# Autodesk Inventor assembly: magplate_blank
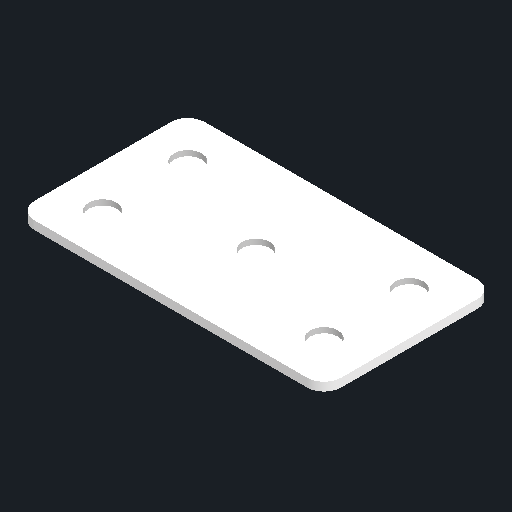
[picture p0: Inventor's stored thumbnail of the model, 512x512]
Saved by Autodesk Inventor 2025 (Build 290162000, 162)
## iProperties
Created: 2024-06-22
Part Number: magplate_blank
Document SubType Name: Assembly
Designer: AdminForWorker
Title: magplate_blank v6
Author: AdminForWorker
## Documents named in this file (6)
- D:\vex_robotics_high_stakes\hardware\cad\magplate_final\magplate.iam
- magplate.iam
- D:\vex_robotics_high_stakes\hardware\cad\magplate_final\Component2.ipt
- D:\vex_robotics_high_stakes\hardware\cad\magplate_final\Component4.ipt
- D:\vex_robotics_high_stakes\hardware\cad\magplate_final\Part8.ipt
- D:\vex_robotics_high_stakes\hardware\cad\magplate_final\Rim.ipt
## Components (4 placed, 4 different names)
1. Component2:1
2. Component4:1
3. Part8 — Flush:1
4. Rim:1 — Flush:1
## Relationships (1: Flush 1)
- Flush:1: Part8 ↔ Rim:1
